# Autodesk Inventor assembly: Actual Robot
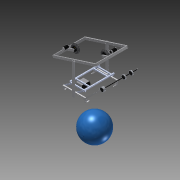
[picture p0: Inventor's stored thumbnail of the model, 180x180]
Saved by Autodesk Inventor 2014 (Build 180170000, 170)
## iProperties
Created: 2014-01-18
Part Number: Actual Robot
Document SubType Name: Assembly
Designer: Paul
Author: Paul
## Documents named in this file (34)
- C:\4859cad\Robot\Actual Robot\Actual Robot.iam
- C:\4859cad\Robot\Drivetrain\Drivetrain Assembly\FrameAssembly .iam
- C:\4859cad\Robot\Structure\Frame Assembly\1x1 tube 22in.ipt
- C:\4859cad\Robot\Structure\Frame Assembly\2x1 Tube 24in.ipt
- C:\4859cad\Robot\Structure\Imported Components\L Guesset\L Guesset.ipt
- C:\4859cad\Robot\Actual Robot\Acquire\Corner Gusset.ipt
- C:\4859cad\Robot\Structure\Frame Assembly\1x1 tube 3 in.ipt
- C:\4859cad\Robot\KOP STEP\Electrical\Imported Components\ELEC_Battery_NP18-12B.iam\ELEC_Battery_NP18-12B.iam.iam
- C:\4859cad\Robot\Structure\Imported Components\T Guesset\T Guesset.ipt
- C:\4859cad\Robot\Structure\Imported Components\End_Cap_Bearing_Mount\End_Cap_Bearing_Mount.ipt
- C:\4859cad\Robot\Structure\Frame Assembly\1x1 tube 23in.ipt
- C:\4859cad\Robot\Actual Robot\Acquire\Real Hex Bearing.ipt
- C:\4859cad\Robot\Actual Robot\Acquire\33 in hex shaft.ipt
- C:\4859cad\Robot\Structure\Frame Assembly\2x1 Tube 43in.ipt
- C:\4859cad\Robot\Structure\Frame Assembly\2x1 Tube 29in.ipt
- C:\4859cad\Robot\Actual Robot\Fly Wheel\Imported Components\PneumaticWheel_am-0970\PneumaticWheel_am-0970.iam
- C:\4859cad\Robot\Actual Robot\Fly Wheel\special hub for flywheels.ipt
- C:\4859cad\Robot\Actual Robot\Fly Wheel\Imported Components\#35 Sprocket 30t\#35 Sprocket 30t.ipt
- C:\4859cad\Robot\Structure\Frame Assembly\2x1 Tube 6in.ipt
- C:\4859cad\Robot\KOP STEP\Drive Base Kit\FIRST Drive Base Wide\Parts\Imported Components\CIM Motor SW.ipt\CIM Motor SW.ipt.ipt
- C:\4859cad\Robot\Actual Robot\Acquire\Round Bearing.ipt
- C:\Users\Paul\Documents\Inventor\Content Center Files\R2014\en-US\ANSI ASME B18.2.1(2)\ANSI_ASME B18.2.1 - 3_8-16 UNC - 6.5(2).ipt
- C:\4859cad\Robot\Actual Robot\Fly Wheel\Imported Components\8mm to .5 hex\8mm to .5 hex.ipt
- C:\4859cad\Robot\Actual Robot\Fly Wheel\Imported Components\#35 Sprocket 15t double\#35 Sprocket 15t double.ipt
- C:\4859cad\Robot\Actual Robot\Fly Wheel\Imported Components\CIM face mount\CIM face mount.ipt
- C:\4859cad\Robot\Actual Robot\Acquire\4 in wheel.iam
- C:\4859cad\Robot\Actual Robot\Acquire\500EX Hex wheel Hub.ipt
- C:\4859cad\Robot\Structure\Frame Assembly\1x1 tube 8 in.ipt
- C:\4859cad\Robot\Structure\Frame Assembly\1x1 tube 7 in.ipt
- C:\4859cad\Robot\Structure\Frame Assembly\1x1 tube 26in.ipt
- C:\4859cad\Robot\Structure\Frame Assembly\1x1 tube 11in.ipt
- C:\4859cad\Robot\Actual Robot\Blue Game Ball.ipt
- ELEC_Battery_NP18-12B.iam
- CIM Motor SW.ipt
## Components (75 placed, 31 different names)
1. FrameAssembly :1 [sub-assembly] — Mate:1, Flush:3, Flush:4, Mate:2, Flush:5, Flush:6, Flush:12, Flush:14, Mate:10, Mate:12, Mate:13, Mate:14, Mate:17, Mate:23, Mate:24, Mate:29, Mate:30, Mate:33, Mate:41, Mate:42, Mate:43, Mate:50, Mate:51
2. 2x1 Tube 24in:1 — Mate:1, Flush:3, Flush:5, Mate:9, Mate:102, Mate:103
3. 2x1 Tube 24in:2 — Flush:4, Mate:2, Flush:6, Mate:104, Mate:105
4. L Guesset:2 — Mate:25, Mate:26, Mate:27, Mate:28
5. Corner Gusset:1 — Mate:12, Mate:13, Mate:14
6. 1x1 tube 22in:1 — Flush:12, Mate:9, Flush:13, Mate:11, Mate:25, Mate:26, Mate:28, Mate:81, Mate:177, Mate:205, Mate:210, Mate:225, Mate:236
7. 1x1 tube 22in:2 — Mate:74, Flush:19, Mate:79, Mate:176, Flush:51, Mate:208, Mate:223, Mate:224, Mate:226
8. 1x1 tube 3 in:1 — Flush:13, Flush:14, Mate:10, Mate:11, Mate:27
9. Corner Gusset:2 — Mate:17, Mate:18, Mate:23, Mate:24
10. 1x1 tube 3 in:2 — Mate:18
11. Corner Gusset:3 — Mate:29, Mate:30, Mate:31, Mate:32, Mate:33, Mate:34
12. Corner Gusset:4 — Mate:41, Mate:42, Mate:43, Mate:44, Mate:45, Mate:46
13. 1x1 tube 3 in:3 — Mate:31, Mate:32, Mate:34, Flush:51
14. 1x1 tube 3 in:5 — Mate:44, Mate:45, Mate:46, Mate:74, Flush:19
15. ELEC_Battery_NP18-12B.iam:1 [sub-assembly] — Mate:50, Mate:51
16. End_Cap_Bearing_Mount:1 — Mate:77, Mate:83, Mate:84, Mate:94, Mate:96
17. End_Cap_Bearing_Mount:2 — Mate:78, Mate:89, Mate:90, Mate:92, Mate:97
18. End_Cap_Bearing_Mount:3 — Mate:75, Mate:85, Mate:86, Mate:91, Mate:95
19. End_Cap_Bearing_Mount:4 — Mate:76, Mate:87, Mate:88, Mate:93, Mate:98
20. 1x1 tube 23in:1 — Mate:76, Mate:78, Mate:79, Mate:87, Mate:88, Mate:89, Mate:90, Mate:176
21. 1x1 tube 23in:2 — Mate:75, Mate:77, Mate:81, Mate:83, Mate:84, Mate:85, Mate:86, Flush:23, Mate:177
22. Real Hex Bearing:1 — Mate:91, Mate:95, Flush:20, Flush:22, Mate:172, Mate:175
23. Real Hex Bearing:2 — Mate:92, Mate:97, Flush:21, Mate:173, Mate:174
24. Real Hex Bearing:3 — Mate:93, Mate:98, Flush:21, Flush:22, Mate:101
25. Real Hex Bearing:4 — Mate:94, Mate:96, Mate:99, Mate:100, Flush:20
26. 33 in hex shaft:1 — Mate:99, Mate:100, Mate:101, Flush:23
27. 2x1 Tube 43in:1 — Mate:104, Mate:105, Flush:26, Flush:27, Flush:28, Mate:107, Flush:30, Flush:31
28. 2x1 Tube 43in:2 — Mate:102, Mate:103, Mate:106, Flush:24, Flush:25, Flush:29
29. 2x1 Tube 29in:1 — Flush:28, Flush:29, Mate:107, Flush:30, Flush:31, Flush:33, Flush:35, Mate:109, Mate:111, Mate:160, Flush:44
30. 2x1 Tube 29in:2 — Mate:106, Flush:24, Flush:25, Flush:26, Flush:27, Mate:108, Flush:32, Flush:34, Mate:110, Mate:121, Mate:122, Mate:127, Mate:128, Mate:129, Mate:130, Mate:185, Flush:46
31. PneumaticWheel_am-0970:1 [sub-assembly] — Mate:119, Mate:131, Mate:132, Flush:36, Mate:133, Flush:37, Mate:137
32. PneumaticWheel_am-0970:2 [sub-assembly] — Flush:40, Flush:41, Mate:143, Mate:144, Mate:146, Mate:147, Mate:148
33. 2x1 Tube 6in:1 — Mate:108, Flush:32, Mate:123, Mate:124, Flush:39
34. 2x1 Tube 6in:2 — Flush:34, Mate:110, Mate:125, Mate:126, Mate:134, Mate:135, Mate:140, Flush:38, Flush:47
35. 2x1 Tube 6in:3 — Flush:33, Mate:111, Mate:141, Mate:142, Flush:39, Mate:152, Flush:42
36. 2x1 Tube 6in:4 — Flush:35, Mate:109, Flush:38, Mate:222
37. CIM Motor SW.ipt:1 — Mate:153, Mate:156, Mate:157, Mate:158, Mate:159
38. #35 Sprocket 30t:1 — Mate:116, Mate:138, Mate:139, Mate:140
39. special hub for flywheels:1 — Mate:116, Mate:119, Mate:131, Mate:137, Mate:138, Mate:139
40. T Guesset:5 — Mate:121, Mate:123, Mate:124, Mate:129, Mate:130
41. T Guesset:6 — Mate:122, Mate:125, Mate:126, Mate:127, Mate:128
42. Round Bearing:1 — Mate:133, Flush:37
43. Round Bearing:2 — Mate:132, Flush:36, Mate:136
44. Hex Bolt - Inch 3/8-16 UNC - 6.5:1 — Mate:134, Mate:135, Mate:136
45. Hex Bolt - Inch 3/8-16 UNC - 6.5:2 — Mate:141, Mate:142, Mate:145
46. Round Bearing:3 — Flush:41, Mate:143
47. Round Bearing:4 — Flush:40, Mate:144, Mate:145, Mate:222
48. #35 Sprocket 30t:2 — Mate:149, Mate:150, Mate:151, Mate:152, Rotation:1
49. special hub for flywheels:2 — Mate:146, Mate:147, Mate:148, Mate:149, Mate:150, Mate:151
50. 8mm to .5 hex:2 — Mate:153, Mate:154, Mate:155, Mate:156, Flush:43
51. #35 Sprocket 15t double:1 — Mate:154, Mate:155, Flush:43, Rotation:1
52. CIM face mount:1 — Mate:157, Mate:158, Mate:159, Mate:160, Flush:42, Flush:44
53. 4 in wheel:1 [sub-assembly] — Mate:161, Mate:165, Rotation:2, Mate:175
54. 500EX Hex wheel Hub:1 — Mate:161, Mate:165, Rotation:2
55. 4 in wheel:2 [sub-assembly]
56. 500EX Hex wheel Hub:2 — Mate:172
57. 4 in wheel:3 [sub-assembly] — Mate:173
58. 500EX Hex wheel Hub:3
59. 4 in wheel:4 [sub-assembly] — Mate:174
60. 500EX Hex wheel Hub:4
61. CIM Motor SW.ipt:2
62. 8mm to .5 hex:3
63. #35 Sprocket 15t double:2
64. CIM face mount:2 — Mate:185, Flush:46, Flush:47
65. 1x1 tube 8 in:1 — Mate:223, Mate:224, Mate:231, Mate:235
66. 1x1 tube 7 in:2 — Mate:228, Mate:231, Mate:232, Mate:233, Mate:234, Mate:235
67. 1x1 tube 8 in:2 — Mate:208, Mate:226, Mate:234
68. 1x1 tube 8 in:6 — Mate:210, Mate:236
69. 1x1 tube 7 in:6 — Mate:206, Mate:212, Mate:214, Mate:215, Mate:221, Mate:237
70. 1x1 tube 8 in:7 — Mate:205, Mate:206, Mate:225
71. 1x1 tube 26in:1 — Mate:212, Mate:214, Mate:218, Mate:219, Flush:54, Flush:55, Mate:228, Mate:232
72. 1x1 tube 26in:2 — Mate:215, Mate:233, Mate:237
73. 1x1 tube 11in:1 — Mate:218, Flush:55, Mate:220, Mate:221
74. 1x1 tube 11in:2 — Mate:219, Flush:54, Mate:220
75. Blue Game Ball:1
## Relationships (200: Mate 156, Flush 39, RelateRotation 5)
- Mate:1: FrameAssembly :1 ↔ 2x1 Tube 24in:1
- Flush:3: FrameAssembly :1 ↔ 2x1 Tube 24in:1
- Flush:4: FrameAssembly :1 ↔ 2x1 Tube 24in:2
- Mate:2: FrameAssembly :1 ↔ 2x1 Tube 24in:2
- Flush:5 (254 mm): FrameAssembly :1 ↔ 2x1 Tube 24in:1
- Flush:6 (254 mm): FrameAssembly :1 ↔ 2x1 Tube 24in:2
- Flush:12: FrameAssembly :1 ↔ 1x1 tube 22in:1
- Mate:9: 2x1 Tube 24in:1 ↔ 1x1 tube 22in:1
- Flush:13: 1x1 tube 22in:1 ↔ 1x1 tube 3 in:1
- Flush:14: FrameAssembly :1 ↔ 1x1 tube 3 in:1
- Mate:10: FrameAssembly :1 ↔ 1x1 tube 3 in:1
- Mate:11: 1x1 tube 22in:1 ↔ 1x1 tube 3 in:1
- Mate:12: FrameAssembly :1 ↔ Corner Gusset:1
- Mate:13: FrameAssembly :1 ↔ Corner Gusset:1
- Mate:14: FrameAssembly :1 ↔ Corner Gusset:1
- Mate:17: FrameAssembly :1 ↔ Corner Gusset:2
- Mate:18: Corner Gusset:2 ↔ 1x1 tube 3 in:2
- Mate:23: FrameAssembly :1 ↔ Corner Gusset:2
- Mate:24: FrameAssembly :1 ↔ Corner Gusset:2
- Mate:25: L Guesset:2 ↔ 1x1 tube 22in:1
- Mate:26: L Guesset:2 ↔ 1x1 tube 22in:1
- Mate:27: L Guesset:2 ↔ 1x1 tube 3 in:1
- Mate:28: L Guesset:2 ↔ 1x1 tube 22in:1
- Mate:29: FrameAssembly :1 ↔ Corner Gusset:3
- Mate:30: FrameAssembly :1 ↔ Corner Gusset:3
- Mate:31: Corner Gusset:3 ↔ 1x1 tube 3 in:3
- Mate:32: Corner Gusset:3 ↔ 1x1 tube 3 in:3
- Mate:33: FrameAssembly :1 ↔ Corner Gusset:3
- Mate:34: Corner Gusset:3 ↔ 1x1 tube 3 in:3
- Mate:41: FrameAssembly :1 ↔ Corner Gusset:4
- Mate:42: FrameAssembly :1 ↔ Corner Gusset:4
- Mate:43: FrameAssembly :1 ↔ Corner Gusset:4
- Mate:44: Corner Gusset:4 ↔ 1x1 tube 3 in:5
- Mate:45: Corner Gusset:4 ↔ 1x1 tube 3 in:5
- Mate:46: Corner Gusset:4 ↔ 1x1 tube 3 in:5
- Mate:50: FrameAssembly :1 ↔ ELEC_Battery_NP18-12B.iam:1
- Mate:51: FrameAssembly :1 ↔ ELEC_Battery_NP18-12B.iam:1
- Mate:74: 1x1 tube 22in:2 ↔ 1x1 tube 3 in:5
- Flush:19: 1x1 tube 22in:2 ↔ 1x1 tube 3 in:5
- Mate:75: End_Cap_Bearing_Mount:3 ↔ 1x1 tube 23in:2
- Mate:76: End_Cap_Bearing_Mount:4 ↔ 1x1 tube 23in:1
- Mate:77: End_Cap_Bearing_Mount:1 ↔ 1x1 tube 23in:2
- Mate:78: End_Cap_Bearing_Mount:2 ↔ 1x1 tube 23in:1
- Mate:79: 1x1 tube 22in:2 ↔ 1x1 tube 23in:1
- Mate:81: 1x1 tube 22in:1 ↔ 1x1 tube 23in:2
- Mate:83: End_Cap_Bearing_Mount:1 ↔ 1x1 tube 23in:2
- Mate:84: End_Cap_Bearing_Mount:1 ↔ 1x1 tube 23in:2
- Mate:85: End_Cap_Bearing_Mount:3 ↔ 1x1 tube 23in:2
- Mate:86: End_Cap_Bearing_Mount:3 ↔ 1x1 tube 23in:2
- Mate:87: End_Cap_Bearing_Mount:4 ↔ 1x1 tube 23in:1
- Mate:88: End_Cap_Bearing_Mount:4 ↔ 1x1 tube 23in:1
- Mate:89: End_Cap_Bearing_Mount:2 ↔ 1x1 tube 23in:1
- Mate:90: End_Cap_Bearing_Mount:2 ↔ 1x1 tube 23in:1
- Mate:91: End_Cap_Bearing_Mount:3 ↔ Real Hex Bearing:1
- Mate:92: End_Cap_Bearing_Mount:2 ↔ Real Hex Bearing:2
- Mate:93: End_Cap_Bearing_Mount:4 ↔ Real Hex Bearing:3
- Mate:94: End_Cap_Bearing_Mount:1 ↔ Real Hex Bearing:4
- Mate:95: End_Cap_Bearing_Mount:3 ↔ Real Hex Bearing:1
- Mate:96: End_Cap_Bearing_Mount:1 ↔ Real Hex Bearing:4
- Mate:97: End_Cap_Bearing_Mount:2 ↔ Real Hex Bearing:2
- Mate:98: End_Cap_Bearing_Mount:4 ↔ Real Hex Bearing:3
- Mate:99: Real Hex Bearing:4 ↔ 33 in hex shaft:1
- Mate:100: Real Hex Bearing:4 ↔ 33 in hex shaft:1
- Flush:20: Real Hex Bearing:1 ↔ Real Hex Bearing:4
- Flush:21: Real Hex Bearing:2 ↔ Real Hex Bearing:3
- Flush:22: Real Hex Bearing:1 ↔ Real Hex Bearing:3
- Mate:101: Real Hex Bearing:3 ↔ 33 in hex shaft:1
- Flush:23: 1x1 tube 23in:2 ↔ 33 in hex shaft:1
- Mate:102: 2x1 Tube 24in:1 ↔ 2x1 Tube 43in:2
- Mate:103: 2x1 Tube 24in:1 ↔ 2x1 Tube 43in:2
- Mate:104: 2x1 Tube 24in:2 ↔ 2x1 Tube 43in:1
- Mate:105: 2x1 Tube 24in:2 ↔ 2x1 Tube 43in:1
- Mate:106: 2x1 Tube 43in:2 ↔ 2x1 Tube 29in:2
- Flush:24: 2x1 Tube 43in:2 ↔ 2x1 Tube 29in:2
- Flush:25: 2x1 Tube 43in:2 ↔ 2x1 Tube 29in:2
- Flush:26: 2x1 Tube 43in:1 ↔ 2x1 Tube 29in:2
- Flush:27: 2x1 Tube 43in:1 ↔ 2x1 Tube 29in:2
- Flush:28: 2x1 Tube 43in:1 ↔ 2x1 Tube 29in:1
- Flush:29: 2x1 Tube 43in:2 ↔ 2x1 Tube 29in:1
- Mate:107: 2x1 Tube 43in:1 ↔ 2x1 Tube 29in:1
- Flush:30: 2x1 Tube 43in:1 ↔ 2x1 Tube 29in:1
- Flush:31: 2x1 Tube 43in:1 ↔ 2x1 Tube 29in:1
- Mate:108: 2x1 Tube 29in:2 ↔ 2x1 Tube 6in:1
- Flush:32: 2x1 Tube 29in:2 ↔ 2x1 Tube 6in:1
- Flush:33: 2x1 Tube 29in:1 ↔ 2x1 Tube 6in:3
- Flush:34: 2x1 Tube 29in:2 ↔ 2x1 Tube 6in:2
- Flush:35: 2x1 Tube 29in:1 ↔ 2x1 Tube 6in:4
- Mate:109: 2x1 Tube 29in:1 ↔ 2x1 Tube 6in:4
- Mate:110: 2x1 Tube 29in:2 ↔ 2x1 Tube 6in:2
- Mate:111: 2x1 Tube 29in:1 ↔ 2x1 Tube 6in:3
- Mate:116: #35 Sprocket 30t:1 ↔ special hub for flywheels:1
- Mate:119: PneumaticWheel_am-0970:1 ↔ special hub for flywheels:1
- Mate:121: 2x1 Tube 29in:2 ↔ T Guesset:5
- Mate:122: 2x1 Tube 29in:2 ↔ T Guesset:6
- Mate:123: 2x1 Tube 6in:1 ↔ T Guesset:5
- Mate:124: 2x1 Tube 6in:1 ↔ T Guesset:5
- Mate:125: 2x1 Tube 6in:2 ↔ T Guesset:6
- Mate:126: 2x1 Tube 6in:2 ↔ T Guesset:6
- Mate:127: 2x1 Tube 29in:2 ↔ T Guesset:6
- Mate:128: 2x1 Tube 29in:2 ↔ T Guesset:6
- Mate:129: 2x1 Tube 29in:2 ↔ T Guesset:5
- Mate:130: 2x1 Tube 29in:2 ↔ T Guesset:5
- Mate:131: PneumaticWheel_am-0970:1 ↔ special hub for flywheels:1
- Mate:132: PneumaticWheel_am-0970:1 ↔ Round Bearing:2
- Flush:36: PneumaticWheel_am-0970:1 ↔ Round Bearing:2
- Mate:133: PneumaticWheel_am-0970:1 ↔ Round Bearing:1
- Flush:37: PneumaticWheel_am-0970:1 ↔ Round Bearing:1
- Mate:134: 2x1 Tube 6in:2 ↔ Hex Bolt - Inch 3/8-16 UNC - 6.5:1
- Mate:135: 2x1 Tube 6in:2 ↔ Hex Bolt - Inch 3/8-16 UNC - 6.5:1
- Mate:136: Round Bearing:2 ↔ Hex Bolt - Inch 3/8-16 UNC - 6.5:1
- Mate:137: PneumaticWheel_am-0970:1 ↔ special hub for flywheels:1
- Mate:138: #35 Sprocket 30t:1 ↔ special hub for flywheels:1
- Mate:139: #35 Sprocket 30t:1 ↔ special hub for flywheels:1
- Mate:140 (12.7 mm): 2x1 Tube 6in:2 ↔ #35 Sprocket 30t:1
- Mate:141: 2x1 Tube 6in:3 ↔ Hex Bolt - Inch 3/8-16 UNC - 6.5:2
- Mate:142: 2x1 Tube 6in:3 ↔ Hex Bolt - Inch 3/8-16 UNC - 6.5:2
- Flush:38: 2x1 Tube 6in:2 ↔ 2x1 Tube 6in:4
- Flush:39: 2x1 Tube 6in:1 ↔ 2x1 Tube 6in:3
- Flush:40: PneumaticWheel_am-0970:2 ↔ Round Bearing:4
- Flush:41: PneumaticWheel_am-0970:2 ↔ Round Bearing:3
- Mate:143: PneumaticWheel_am-0970:2 ↔ Round Bearing:3
- Mate:144: PneumaticWheel_am-0970:2 ↔ Round Bearing:4
- Mate:145: Hex Bolt - Inch 3/8-16 UNC - 6.5:2 ↔ Round Bearing:4
- Mate:146: PneumaticWheel_am-0970:2 ↔ special hub for flywheels:2
- Mate:147: PneumaticWheel_am-0970:2 ↔ special hub for flywheels:2
- Mate:148: PneumaticWheel_am-0970:2 ↔ special hub for flywheels:2
- Mate:149: #35 Sprocket 30t:2 ↔ special hub for flywheels:2
- Mate:150: #35 Sprocket 30t:2 ↔ special hub for flywheels:2
- Mate:151: #35 Sprocket 30t:2 ↔ special hub for flywheels:2
- Mate:152 (12.7 mm): 2x1 Tube 6in:3 ↔ #35 Sprocket 30t:2
- Mate:153: CIM Motor SW.ipt:1 ↔ 8mm to .5 hex:2
- Mate:154: 8mm to .5 hex:2 ↔ #35 Sprocket 15t double:1
- Mate:155: 8mm to .5 hex:2 ↔ #35 Sprocket 15t double:1
- Mate:156 (2.54 mm): CIM Motor SW.ipt:1 ↔ 8mm to .5 hex:2
- Mate:157: CIM Motor SW.ipt:1 ↔ CIM face mount:1
- Mate:158: CIM Motor SW.ipt:1 ↔ CIM face mount:1
- Mate:159: CIM Motor SW.ipt:1 ↔ CIM face mount:1
- Mate:160: 2x1 Tube 29in:1 ↔ CIM face mount:1
- Flush:42: 2x1 Tube 6in:3 ↔ CIM face mount:1
- Flush:43 (6.35 mm): 8mm to .5 hex:2 ↔ #35 Sprocket 15t double:1
- Flush:44: 2x1 Tube 29in:1 ↔ CIM face mount:1
- Rotation:1 [RelateRotation] (0.5 ul): #35 Sprocket 30t:2 ↔ #35 Sprocket 15t double:1
- Mate:161: 4 in wheel:1 ↔ 500EX Hex wheel Hub:1
- Mate:165: 4 in wheel:1 ↔ 500EX Hex wheel Hub:1
- Rotation:2 [RelateRotation] (1 ul): 4 in wheel:1 ↔ 500EX Hex wheel Hub:1
- [Mate]: 4 in wheel:2 ↔ 500EX Hex wheel Hub:2
- [Mate]: 4 in wheel:2 ↔ 500EX Hex wheel Hub:2
- [RelateRotation] (1 ul): 4 in wheel:2 ↔ 500EX Hex wheel Hub:2
- [Mate]: 4 in wheel:3 ↔ 500EX Hex wheel Hub:3
- [Mate]: 4 in wheel:3 ↔ 500EX Hex wheel Hub:3
- [RelateRotation] (1 ul): 4 in wheel:3 ↔ 500EX Hex wheel Hub:3
- [Mate]: 4 in wheel:4 ↔ 500EX Hex wheel Hub:4
- [Mate]: 4 in wheel:4 ↔ 500EX Hex wheel Hub:4
- [RelateRotation] (1 ul): 4 in wheel:4 ↔ 500EX Hex wheel Hub:4
- Mate:172: Real Hex Bearing:1 ↔ 500EX Hex wheel Hub:2
- Mate:173: Real Hex Bearing:2 ↔ 4 in wheel:3
- Mate:174: Real Hex Bearing:2 ↔ 4 in wheel:4
- Mate:175: Real Hex Bearing:1 ↔ 4 in wheel:1
- Mate:176: 1x1 tube 22in:2 ↔ 1x1 tube 23in:1
- Mate:177: 1x1 tube 22in:1 ↔ 1x1 tube 23in:2
- [Mate]: CIM Motor SW.ipt:2 ↔ 8mm to .5 hex:3
- [Mate]: 8mm to .5 hex:3 ↔ #35 Sprocket 15t double:2
- [Mate]: 8mm to .5 hex:3 ↔ #35 Sprocket 15t double:2
- [Mate] (2.54 mm): CIM Motor SW.ipt:2 ↔ 8mm to .5 hex:3
- [Mate]: CIM Motor SW.ipt:2 ↔ CIM face mount:2
- [Mate]: CIM Motor SW.ipt:2 ↔ CIM face mount:2
- [Mate]: CIM Motor SW.ipt:2 ↔ CIM face mount:2
- [Flush] (6.35 mm): 8mm to .5 hex:3 ↔ #35 Sprocket 15t double:2
- Mate:185: 2x1 Tube 29in:2 ↔ CIM face mount:2
- Flush:46: 2x1 Tube 29in:2 ↔ CIM face mount:2
- Flush:47: 2x1 Tube 6in:2 ↔ CIM face mount:2
- [Mate]: 1x1 tube 8 in:6 ↔ 1x1 tube 7 in:6
- [Mate]: 1x1 tube 7 in:6 ↔ 1x1 tube 8 in:7
- Flush:51: 1x1 tube 22in:2 ↔ 1x1 tube 3 in:3
- Mate:205: 1x1 tube 22in:1 ↔ 1x1 tube 8 in:7
- Mate:206: 1x1 tube 7 in:6 ↔ 1x1 tube 8 in:7
- Mate:208: 1x1 tube 22in:2 ↔ 1x1 tube 8 in:2
- Mate:210: 1x1 tube 22in:1 ↔ 1x1 tube 8 in:6
- Mate:212: 1x1 tube 7 in:6 ↔ 1x1 tube 26in:1
- Mate:214: 1x1 tube 7 in:6 ↔ 1x1 tube 26in:1
- Mate:215: 1x1 tube 7 in:6 ↔ 1x1 tube 26in:2
- Mate:218: 1x1 tube 26in:1 ↔ 1x1 tube 11in:1
- Mate:219: 1x1 tube 26in:1 ↔ 1x1 tube 11in:2
- Flush:54: 1x1 tube 26in:1 ↔ 1x1 tube 11in:2
- Flush:55: 1x1 tube 26in:1 ↔ 1x1 tube 11in:1
- Mate:220 (406.4 mm): 1x1 tube 11in:1 ↔ 1x1 tube 11in:2
- Mate:221 (88.9 mm): 1x1 tube 7 in:6 ↔ 1x1 tube 11in:1
- Mate:222: 2x1 Tube 6in:4 ↔ Round Bearing:4
- Mate:223: 1x1 tube 22in:2 ↔ 1x1 tube 8 in:1
- Mate:224: 1x1 tube 22in:2 ↔ 1x1 tube 8 in:1
- Mate:225: 1x1 tube 22in:1 ↔ 1x1 tube 8 in:7
- Mate:226: 1x1 tube 22in:2 ↔ 1x1 tube 8 in:2
- Mate:228: 1x1 tube 7 in:2 ↔ 1x1 tube 26in:1
- Mate:231: 1x1 tube 8 in:1 ↔ 1x1 tube 7 in:2
- Mate:232: 1x1 tube 7 in:2 ↔ 1x1 tube 26in:1
- Mate:233: 1x1 tube 7 in:2 ↔ 1x1 tube 26in:2
- Mate:234: 1x1 tube 7 in:2 ↔ 1x1 tube 8 in:2
- Mate:235: 1x1 tube 8 in:1 ↔ 1x1 tube 7 in:2
- Mate:236: 1x1 tube 22in:1 ↔ 1x1 tube 8 in:6
- Mate:237: 1x1 tube 7 in:6 ↔ 1x1 tube 26in:2
## Named parameters: d304_d298 = 0 mm, d305_d302 = 0 mm, d306_d303 = 1, d307_d298 = 0 mm, d308_d302 = 0 mm, d309_d303 = 1, d310_d298 = 0 mm, d311_d302 = 0 mm, d312_d303 = 1, d319_d284 = 0 mm, d320_d286 = 0 mm, d321_d287 = 0 mm, d322_d288 = 2.54 mm, d323_d289 = 0 mm, d324_d290 = 0 mm, d325_d291 = 0 mm, d326_d294 = 6.35 mm, d373_d366 = 0 mm, d374_d368 = 0 mm
